# Autodesk Inventor assembly: VOORWIEL_TOTAAL
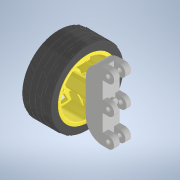
[picture p0: Inventor's stored thumbnail of the model, 180x180]
Saved by Autodesk Inventor 2022 (Build 260153000, 153)
## iProperties
Created: 2021-12-16
Part Number: VOORWIEL_TOTAAL
Document SubType Name: Assembly
Designer: keemi
Author: keemi
## Documents named in this file (4)
- C:\Users\keemi\OneDrive\Bureaublad\repo's\projecten\Auto\modellen\inventor\auto moddel\VOORWIEL_TOTAAL.iam
- C:\Users\keemi\OneDrive\Bureaublad\repo's\projecten\Auto\modellen\inventor\stuur_arm v2.ipt
- C:\Users\keemi\OneDrive\Bureaublad\repo's\projecten\Auto\modellen\inventor\wheel-arduino-1.snapshot.2\Wheel ALL.ipt
- C:\Users\keemi\OneDrive\Bureaublad\repo's\projecten\Auto\modellen\inventor\draaiarm voorwielen.ipt
## Components (3 placed, 3 different names)
1. stuur_arm v2:1 — Mate:1, Mate:2
2. Wheel ALL:1 — Mate:3
3. draaiarm voorwielen:1 — Mate:1, Mate:2, Mate:3
## Relationships (3: Mate 3)
- Mate:1: stuur_arm v2:1 ↔ draaiarm voorwielen:1
- Mate:2: stuur_arm v2:1 ↔ draaiarm voorwielen:1
- Mate:3: Wheel ALL:1 ↔ draaiarm voorwielen:1
